# Autodesk Inventor assembly: RailOnBreadBoard
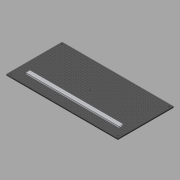
[picture p0: Inventor's stored thumbnail of the model, 180x180]
Saved by Autodesk Inventor 2018 (Build 220112000, 112)
## iProperties
Created: 2018-09-17
Part Number: RailOnBreadBoard
Document SubType Name: Assembly
Designer: Robert Campbell
Author: Robert Campbell
## Documents named in this file (3)
- \\Mac\Home\Dropbox (UCL - SWC)\work\WorkDocs\MF_BenchOptics\CAD_files\RailOnBreadBoard.iam
- \\Mac\Home\Dropbox (UCL - SWC)\work\WorkDocs\MF_BenchOptics\CAD_files\MB60120_M-Solidworks.ipt
- \\Mac\Home\Dropbox (UCL - SWC)\work\WorkDocs\MF_BenchOptics\CAD_files\XT66DP-1000-Solidworks.ipt
## Components (2 placed, 2 different names)
1. MB60120_M-Solidworks:1 — Mate:1
2. XT66DP-1000-Solidworks:1 — Mate:1
## Relationships (1: Mate 1)
- Mate:1: MB60120_M-Solidworks:1 ↔ XT66DP-1000-Solidworks:1
